# Autodesk Inventor assembly: WCS-01
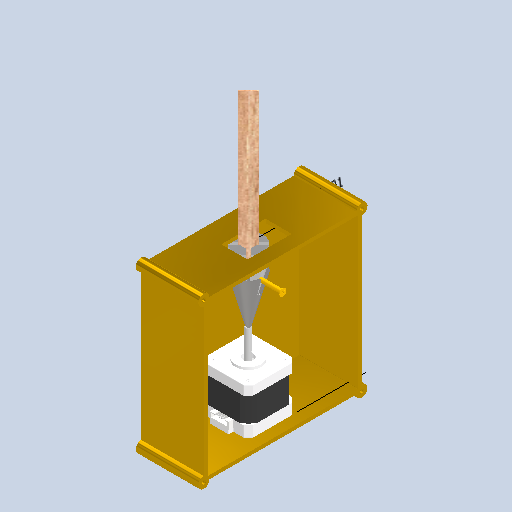
[picture p0: Inventor's stored thumbnail of the model, 512x512]
Saved by Autodesk Inventor 2022 (Build 260153000, 153)
## iProperties
Company: El Camino College
Created: 2023-06-01
Part Number: WCS-01
Document SubType Name: Assembly
Designer: Edgar Tejada
Mass: 510.99 g
Surface Area: 1355.27 cm^2
Volume: 232.006 cm^3
Density: 2.20248 g/cm^3
Description: Subassembly for Cutting Wood Wicks
Author: Edgar Tejada
Title: Wood Cutting Subassembly
## Documents named in this file (7)
- G:\Documents\Inventor HW\Hexagonal_Hive\Wick_Cutting_Sub\Wick-Cutting_Sub.iam
- G:\Documents\Inventor HW\Hexagonal_Hive\Wick_Cutting_Sub\NEMA17.ipt
- G:\Documents\Inventor HW\Hexagonal_Hive\Wick_Cutting_Sub\Collet_Cone.ipt
- G:\Documents\Inventor HW\Hexagonal_Hive\Wick_Cutting_Sub\Collet_Wooden_Wick.ipt
- G:\Documents\Inventor HW\Hexagonal_Hive\Wick_Cutting_Sub\Wood_Wick.ipt
- G:\Documents\Inventor HW\Hexagonal_Hive\Provided_Screws_ANSI B18.6.3 - 6-32 UNC - 2(32).ipt
- G:\Documents\Inventor HW\Hexagonal_Hive\Wick_Cutting_Sub\Panel_Shell.ipt
## Components (6 placed, 6 different names)
1. NEMA17:1 — Insert:1, Insert:2, Mate:2, Angle:3, Mate:4, Mate:6
2. Collet_Cone:1 — Insert:1, Angle:2, Mate:7
3. Collet_Wooden_Wick:1 — Insert:2, Mate:1, Angle:1, Mate:3
4. Wood_Wick:1 — Mate:2, Angle:1, Mate:3
5. Cross Recessed 100° Flat Countersunk Head Machine Screw - Type I - Inch 6-32 UNC x 1:1 — Mate:1, Angle:2, Mate:5
6. Panel_Shell:1 — Angle:3, Mate:4, Mate:5, Mate:6, Mate:7
## Relationships (12: Mate 7, Angle 3, Insert 2)
- Insert:1: NEMA17:1 ↔ Collet_Cone:1
- Insert:2 (25.4 mm): NEMA17:1 ↔ Collet_Wooden_Wick:1
- Mate:1: Collet_Wooden_Wick:1 ↔ Cross Recessed 100° Flat Countersunk Head Machine Screw - Type I - Inch 6-32 UNC x 1:1
- Mate:2 (71.12 mm): NEMA17:1 ↔ Wood_Wick:1
- Angle:1 (0 deg): Collet_Wooden_Wick:1 ↔ Wood_Wick:1
- Angle:2 (90 deg): Collet_Cone:1 ↔ Cross Recessed 100° Flat Countersunk Head Machine Screw - Type I - Inch 6-32 UNC x 1:1
- Mate:3: Collet_Wooden_Wick:1 ↔ Wood_Wick:1
- Angle:3 (180 deg): NEMA17:1 ↔ Panel_Shell:1
- Mate:4: NEMA17:1 ↔ Panel_Shell:1
- Mate:5: Cross Recessed 100° Flat Countersunk Head Machine Screw - Type I - Inch 6-32 UNC x 1:1 ↔ Panel_Shell:1
- Mate:6: NEMA17:1 ↔ Panel_Shell:1
- Mate:7: Collet_Cone:1 ↔ Panel_Shell:1
